# Autodesk Inventor assembly: fork_and_mount
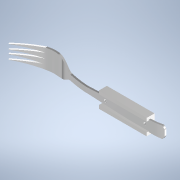
[picture p0: Inventor's stored thumbnail of the model, 180x180]
Saved by Autodesk Inventor 2022 (Build 260153000, 153)
## iProperties
Created: 2022-10-23
Part Number: fork_and_mount
Document SubType Name: Assembly
Designer: Yazawa
Author: Yazawa
## Documents named in this file (3)
- C:\Users\Yazawa\Documents\GitHub\fork\fork_and_mount.iam
- C:\Users\Yazawa\Documents\GitHub\fork\fork.ipt
- C:\Users\Yazawa\Documents\GitHub\fork\forkmount.ipt
## Components (2 placed, 2 different names)
1. fork:1 — メイト:1, メイト:2, 挿入:1
2. forkmount:1 — メイト:1, メイト:2, 挿入:1
## Relationships (3: Mate 2, Insert 1)
- メイト:1 [Mate]: fork:1 ↔ forkmount:1
- メイト:2 [Mate]: fork:1 ↔ forkmount:1
- 挿入:1 [Insert]: fork:1 ↔ forkmount:1
